# Autodesk Inventor assembly: Base_V2
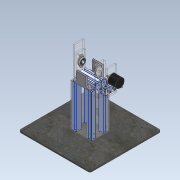
[picture p0: Inventor's stored thumbnail of the model, 180x180]
Saved by Autodesk Inventor 2021.1 (Build 251245010, 245A)
## iProperties
Created: 2023-10-20
Part Number: Base_V2
Document SubType Name: Assembly
Designer: user
Author: user
## Documents named in this file (19)
- F:\College\Semester_10\GP2\2DOF\2DOF_Hover\CAD\Workspaces\Workspace\Base_V2.iam
- F:\College\Semester_10\GP2\2DOF\2DOF_Hover\CAD\Workspaces\Workspace\FlangedBearing8mm.ipt
- F:\College\Semester_10\GP2\2DOF\2DOF_Hover\CAD\Workspaces\Workspace\BaseC_1.ipt
- F:\College\Semester_10\GP2\2DOF\2DOF_Hover\CAD\Workspaces\Workspace\BaseC_2.ipt
- F:\College\Semester_10\GP2\2DOF\2DOF_Hover\CAD\Workspaces\Workspace\BaseC_3.ipt
- F:\College\Semester_10\GP2\2DOF\2DOF_Hover\CAD\Workspaces\Workspace\BaseC_4.ipt
- F:\College\Semester_10\GP2\2DOF\2DOF_Hover\CAD\Workspaces\Workspace\BaseC_5.ipt
- F:\College\Semester_10\GP2\2DOF\2DOF_Hover\CAD\Workspaces\Workspace\Encoder.ipt
- F:\College\Semester_10\GP2\2DOF\2DOF_Hover\CAD\Workspaces\Workspace\BaseC_6.ipt
- F:\College\Semester_10\GP2\2DOF\2DOF_Hover\CAD\Workspaces\Workspace\BaseC_7.ipt
- F:\College\Semester_10\GP2\2DOF\2DOF_Hover\CAD\Workspaces\Workspace\20x20mm V-Slot.ipt
- F:\College\Semester_10\GP2\2DOF\2DOF_Hover\CAD\Workspaces\Workspace\BaseC_8.ipt
- F:\College\Semester_10\GP2\2DOF\2DOF_Hover\CAD\Workspaces\Workspace\BaseC_9.ipt
- F:\College\Semester_10\GP2\2DOF\2DOF_Hover\CAD\Workspaces\Workspace\2020RightAngle.ipt
- F:\College\Semester_10\GP2\2DOF\2DOF_Hover\CAD\Libraries\Content Center Files\en-US\ISO 7045  H\ISO 7045 - M4 x 14 - 4.8 - H - ISO.ipt
- F:\College\Semester_10\GP2\2DOF\2DOF_Hover\CAD\Libraries\Content Center Files\en-US\ISO 4032(2)\ISO 4032 - M4 - ISO.ipt
- F:\College\Semester_10\GP2\2DOF\2DOF_Hover\CAD\Workspaces\Workspace\gard1.ipt
- F:\College\Semester_10\GP2\2DOF\2DOF_Hover\CAD\Workspaces\Workspace\guard 2.ipt
- F:\College\Semester_10\GP2\2DOF\2DOF_Hover\CAD\Workspaces\Workspace\guard3.ipt
## Components (37 placed, 18 different names)
1. FlangedBearing8mm:1 — Mate:65, Mate:66, Mate:67
2. FlangedBearing8mm:2 — Mate:68, Mate:69, Mate:70
3. BaseC_1:1 — Flush:1, Mate:9, Flush:2, Mate:77, Mate:79, Mate:84
4. BaseC_2:1 — Mate:11, Flush:16, Flush:17, Flush:18, Flush:22, Mate:74, Mate:88, Flush:24
5. BaseC_4:1 — Flush:18, Flush:19, Flush:20, Mate:72, Flush:23
6. BaseC_3:1 — Flush:8, Angle:1, Flush:19, Flush:20, Flush:21, Mate:71, Mate:72, Mate:85
7. BaseC_4:2 — Mate:11, Flush:8, Flush:16, Flush:17, Flush:21, Mate:71, Mate:73, Mate:78, Mate:86
8. Encoder:1 — Flush:15, Mate:57
9. BaseC_6:1 — Angle:1, Mate:59, Mate:60, Mate:61, Mate:62, Mate:63, Mate:64, Mate:90, Flush:24
10. BaseC_7:1 — Flush:15, Mate:57, Flush:25, Flush:26, Flush:27, Mate:98, Mate:99, Mate:101, Mate:103, Mate:104, Mate:105, Mate:107
11. 20x20mm V-Slot:1 — Mate:75, Mate:76, Mate:77, Mate:78, Mate:79
12. BaseC_5:1 — Mate:59, Mate:60, Mate:61, Mate:68, Mate:69, Mate:70, Flush:23, Flush:32
13. BaseC_5:2 — Mate:62, Mate:63, Mate:64, Mate:65, Mate:66, Mate:67, Mate:91, Mate:93, Angle:3, Mate:95
14. BaseC_8:1 — Flush:22, Mate:73, Mate:74, Mate:75, Mate:76, Mate:80, Mate:81, Mate:82, Mate:83, Mate:87, Mate:89, Mate:90, Mate:125, Mate:126, Mate:127, Mate:128, Mate:129, Mate:130
15. 20x20mm V-Slot:2 — Mate:80, Mate:82, Mate:85
16. 20x20mm V-Slot:3 — Mate:81, Mate:83, Mate:84, Mate:86
17. 20x20mm V-Slot:4 — Mate:87, Mate:88, Mate:89
18. BaseC_9:1 — Flush:25, Flush:26, Flush:27, Mate:91, Mate:94, Angle:3, Flush:28, Mate:96, Flush:29, Mate:97, Flush:30, Mate:100, Flush:31, Mate:109, Mate:112, Mate:113, Mate:115, Mate:117, Mate:119, Mate:121, Mate:124
19. 2020RightAngle:1 — Mate:93, Mate:94, Flush:28, Mate:118
20. 2020RightAngle:2 — Mate:95, Mate:96, Flush:29, Mate:122
21. 2020RightAngle:3 — Mate:97, Mate:98, Flush:30, Mate:106, Mate:114
22. 2020RightAngle:4 — Mate:99, Mate:100, Flush:31, Mate:102, Mate:110
23. gard1:1 — Flush:32
24. guard 2:1 — Mate:128, Mate:129, Mate:130
25. guard3:1 — Mate:125, Mate:126, Mate:127
26. ISO 7045 H M4 x 14 - 4.8 - H:1 — Mate:101, Mate:102
27. ISO 4032 M4:1 — Mate:103, Mate:104
28. ISO 7045 H M4 x 14 - 4.8 - H:2 — Mate:109, Mate:110, Mate:111
29. ISO 4032 M4:2 — Mate:111, Mate:112
30. ISO 7045 H M4 x 14 - 4.8 - H:3 — Mate:117, Mate:118, Mate:120
31. ISO 4032 M4:3 — Mate:119, Mate:120
32. ISO 7045 H M4 x 14 - 4.8 - H:4 — Mate:105, Mate:106, Mate:108
33. ISO 4032 M4:4 — Mate:107, Mate:108
34. ISO 7045 H M4 x 14 - 4.8 - H:5 — Mate:121, Mate:122, Mate:123
35. ISO 4032 M4:5 — Mate:123, Mate:124
36. ISO 7045 H M4 x 14 - 4.8 - H:6 — Mate:113, Mate:114, Mate:116
37. ISO 4032 M4:6 — Mate:115, Mate:116
## Relationships (97: Mate 74, Flush 21, Angle 2)
- Flush:1: BaseC_1:1
- Mate:9: BaseC_1:1
- Flush:2: BaseC_1:1
- Mate:11: BaseC_2:1 ↔ BaseC_4:2
- Flush:8: BaseC_3:1 ↔ BaseC_4:2
- Angle:1 (0 deg): BaseC_3:1 ↔ BaseC_6:1
- Flush:15: Encoder:1 ↔ BaseC_7:1
- Mate:57: Encoder:1 ↔ BaseC_7:1
- Mate:59: BaseC_6:1 ↔ BaseC_5:1
- Mate:60: BaseC_6:1 ↔ BaseC_5:1
- Mate:61: BaseC_6:1 ↔ BaseC_5:1
- Mate:62: BaseC_6:1 ↔ BaseC_5:2
- Mate:63: BaseC_6:1 ↔ BaseC_5:2
- Mate:64: BaseC_6:1 ↔ BaseC_5:2
- Mate:65: FlangedBearing8mm:1 ↔ BaseC_5:2
- Mate:66: FlangedBearing8mm:1 ↔ BaseC_5:2
- Mate:67: FlangedBearing8mm:1 ↔ BaseC_5:2
- Mate:68: FlangedBearing8mm:2 ↔ BaseC_5:1
- Mate:69: FlangedBearing8mm:2 ↔ BaseC_5:1
- Mate:70: FlangedBearing8mm:2 ↔ BaseC_5:1
- Flush:16: BaseC_2:1 ↔ BaseC_4:2
- Flush:17: BaseC_2:1 ↔ BaseC_4:2
- Flush:18: BaseC_2:1 ↔ BaseC_4:1
- Flush:19: BaseC_4:1 ↔ BaseC_3:1
- Flush:20: BaseC_4:1 ↔ BaseC_3:1
- Flush:21: BaseC_3:1 ↔ BaseC_4:2
- Mate:71: BaseC_3:1 ↔ BaseC_4:2
- Mate:72: BaseC_4:1 ↔ BaseC_3:1
- Flush:22: BaseC_2:1 ↔ BaseC_8:1
- Mate:73: BaseC_4:2 ↔ BaseC_8:1
- Mate:74: BaseC_2:1 ↔ BaseC_8:1
- Mate:75: 20x20mm V-Slot:1 ↔ BaseC_8:1
- Mate:76: 20x20mm V-Slot:1 ↔ BaseC_8:1
- Mate:77: BaseC_1:1 ↔ 20x20mm V-Slot:1
- Mate:78: BaseC_4:2 ↔ 20x20mm V-Slot:1
- Mate:79: BaseC_1:1 ↔ 20x20mm V-Slot:1
- Mate:80: BaseC_8:1 ↔ 20x20mm V-Slot:2
- Mate:81: BaseC_8:1 ↔ 20x20mm V-Slot:3
- Mate:82: BaseC_8:1 ↔ 20x20mm V-Slot:2
- Mate:83: BaseC_8:1 ↔ 20x20mm V-Slot:3
- Mate:84: BaseC_1:1 ↔ 20x20mm V-Slot:3
- Mate:85: BaseC_3:1 ↔ 20x20mm V-Slot:2
- Mate:86: BaseC_4:2 ↔ 20x20mm V-Slot:3
- Mate:87: BaseC_8:1 ↔ 20x20mm V-Slot:4
- Mate:88: BaseC_2:1 ↔ 20x20mm V-Slot:4
- Mate:89: BaseC_8:1 ↔ 20x20mm V-Slot:4
- Flush:23: BaseC_4:1 ↔ BaseC_5:1
- Mate:90: BaseC_6:1 ↔ BaseC_8:1
- Flush:24 (-18 mm): BaseC_2:1 ↔ BaseC_6:1
- Flush:25: BaseC_7:1 ↔ BaseC_9:1
- Flush:26: BaseC_7:1 ↔ BaseC_9:1
- Flush:27: BaseC_7:1 ↔ BaseC_9:1
- Mate:91: BaseC_5:2 ↔ BaseC_9:1
- Mate:93: BaseC_5:2 ↔ 2020RightAngle:1
- Mate:94: BaseC_9:1 ↔ 2020RightAngle:1
- Angle:3 (0 deg): BaseC_5:2 ↔ BaseC_9:1
- Flush:28: BaseC_9:1 ↔ 2020RightAngle:1
- Mate:95: BaseC_5:2 ↔ 2020RightAngle:2
- Mate:96: BaseC_9:1 ↔ 2020RightAngle:2
- Flush:29: BaseC_9:1 ↔ 2020RightAngle:2
- Mate:97: BaseC_9:1 ↔ 2020RightAngle:3
- Mate:98: BaseC_7:1 ↔ 2020RightAngle:3
- Flush:30: BaseC_9:1 ↔ 2020RightAngle:3
- Mate:99: BaseC_7:1 ↔ 2020RightAngle:4
- Mate:100: BaseC_9:1 ↔ 2020RightAngle:4
- Flush:31: BaseC_9:1 ↔ 2020RightAngle:4
- Mate:101: BaseC_7:1 ↔ ISO 7045 H M4 x 14 - 4.8 - H:1
- Mate:102: 2020RightAngle:4 ↔ ISO 7045 H M4 x 14 - 4.8 - H:1
- Mate:103: BaseC_7:1 ↔ ISO 4032 M4:1
- Mate:104: BaseC_7:1 ↔ ISO 4032 M4:1
- Mate:105: BaseC_7:1 ↔ ISO 7045 H M4 x 14 - 4.8 - H:4
- Mate:106: 2020RightAngle:3 ↔ ISO 7045 H M4 x 14 - 4.8 - H:4
- Mate:107: BaseC_7:1 ↔ ISO 4032 M4:4
- Mate:108: ISO 7045 H M4 x 14 - 4.8 - H:4 ↔ ISO 4032 M4:4
- Mate:109: BaseC_9:1 ↔ ISO 7045 H M4 x 14 - 4.8 - H:2
- Mate:110: 2020RightAngle:4 ↔ ISO 7045 H M4 x 14 - 4.8 - H:2
- Mate:111: ISO 7045 H M4 x 14 - 4.8 - H:2 ↔ ISO 4032 M4:2
- Mate:112: BaseC_9:1 ↔ ISO 4032 M4:2
- Mate:113: BaseC_9:1 ↔ ISO 7045 H M4 x 14 - 4.8 - H:6
- Mate:114: 2020RightAngle:3 ↔ ISO 7045 H M4 x 14 - 4.8 - H:6
- Mate:115: BaseC_9:1 ↔ ISO 4032 M4:6
- Mate:116: ISO 7045 H M4 x 14 - 4.8 - H:6 ↔ ISO 4032 M4:6
- Mate:117: BaseC_9:1 ↔ ISO 7045 H M4 x 14 - 4.8 - H:3
- Mate:118: 2020RightAngle:1 ↔ ISO 7045 H M4 x 14 - 4.8 - H:3
- Mate:119: BaseC_9:1 ↔ ISO 4032 M4:3
- Mate:120: ISO 7045 H M4 x 14 - 4.8 - H:3 ↔ ISO 4032 M4:3
- Mate:121: BaseC_9:1 ↔ ISO 7045 H M4 x 14 - 4.8 - H:5
- Mate:122: 2020RightAngle:2 ↔ ISO 7045 H M4 x 14 - 4.8 - H:5
- Mate:123: ISO 7045 H M4 x 14 - 4.8 - H:5 ↔ ISO 4032 M4:5
- Mate:124: BaseC_9:1 ↔ ISO 4032 M4:5
- Flush:32: BaseC_5:1 ↔ gard1:1
- Mate:125: BaseC_8:1 ↔ guard3:1
- Mate:126: BaseC_8:1 ↔ guard3:1
- Mate:127: BaseC_8:1 ↔ guard3:1
- Mate:128: BaseC_8:1 ↔ guard 2:1
- Mate:129: BaseC_8:1 ↔ guard 2:1
- Mate:130: BaseC_8:1 ↔ guard 2:1
